# Autodesk Inventor assembly: PneumaticWheel_am-0970-2
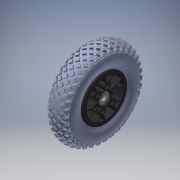
[picture p0: Inventor's stored thumbnail of the model, 180x180]
Saved by Autodesk Inventor 2016 (Build 200138000, 138)
## iProperties
Created: 2011-11-15
Part Number: PneumaticWheel_am-0970-2
Description: STEP AP214
Document SubType Name: Assembly
Designer: gus
Mass: 453.254 g
Surface Area: 2399.32 cm^2
Volume: 453.254 cm^3
Density: 1 g/cm^3
Sending System: SolidWorks 2010
Preprocessor: SwSTEP 2.0
Title: Pneumatic Wheel.STEP
Author: Mark
Revision Number: ANY
## Documents named in this file (7)
- \\Mac\Home\Desktop\2016 robot cad\chassis\PneumaticWheel_am-0970-2.iam
- \\Mac\Home\Desktop\2016 robot cad\chassis\Tire.ipt
- \\Mac\Home\Desktop\2016 robot cad\chassis\Pneumatic Hub.iam
- \\Mac\Home\Desktop\2016 robot cad\chassis\am-0077a-500 Key Hub r2.ipt
- \\Mac\Home\Desktop\2016 robot cad\chassis\spacer.ipt
- \\Mac\Home\Desktop\2016 robot cad\chassis\shaftcollar.ipt
- \\Mac\Home\Desktop\2016 robot cad\chassis\28tsprocket.ipt
## Components (8 placed, 6 different names)
1. Tire_1 — Cylindrical:2, Rigid:1
2. Pneumatic Hub_3 [sub-assembly] — Cylindrical:1, Cylindrical:2, Rigid:1, Mate:1, Mate:2, Mate:3, Rotational:1
3. am-0077a-500 Key Hub r2:1 — Cylindrical:1, Mate:1, Mate:2, Mate:3, Mate:4, Mate:5, Mate:6
4. shaftcollar:1 — Rotational:1
5. shaftcollar:2 — Rotational:2
6. 28tsprocket:1 — Mate:4, Mate:5, Mate:6, Mate:7, Mate:8, Mate:9
7. 28tsprocket:2 — Mate:10, Mate:11, Mate:12
8. spacer:1 — Mate:7, Mate:8, Mate:9, Mate:10, Mate:11, Mate:12, Rotational:2
## Relationships (17: Mate 12, CylindricalJoint 2, RevoluteJoint 2, WeldJoint 1)
- Cylindrical:1: Pneumatic Hub_3 ↔ am-0077a-500 Key Hub r2:1
- Cylindrical:2: Tire_1 ↔ Pneumatic Hub_3
- Rigid:1 [WeldJoint]: Tire_1 ↔ Pneumatic Hub_3
- Mate:1: Pneumatic Hub_3 ↔ am-0077a-500 Key Hub r2:1
- Mate:2: Pneumatic Hub_3 ↔ am-0077a-500 Key Hub r2:1
- Mate:3: Pneumatic Hub_3 ↔ am-0077a-500 Key Hub r2:1
- Rotational:1 [RevoluteJoint]: Pneumatic Hub_3 ↔ shaftcollar:1
- Mate:4: am-0077a-500 Key Hub r2:1 ↔ 28tsprocket:1
- Mate:5: am-0077a-500 Key Hub r2:1 ↔ 28tsprocket:1
- Mate:6: am-0077a-500 Key Hub r2:1 ↔ 28tsprocket:1
- Mate:7: 28tsprocket:1 ↔ spacer:1
- Mate:8: 28tsprocket:1 ↔ spacer:1
- Mate:9: 28tsprocket:1 ↔ spacer:1
- Mate:10: 28tsprocket:2 ↔ spacer:1
- Mate:11: 28tsprocket:2 ↔ spacer:1
- Mate:12: 28tsprocket:2 ↔ spacer:1
- Rotational:2 [RevoluteJoint]: shaftcollar:2 ↔ spacer:1
